# Autodesk Inventor assembly: Cam Follower
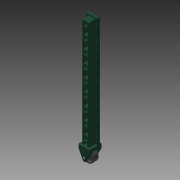
[picture p0: Inventor's stored thumbnail of the model, 180x180]
Saved by Autodesk Inventor 2016 SP2 (Build 200236200, 236)
## iProperties
Created: 2016-05-22
Part Number: Cam Follower
Document SubType Name: Assembly
Designer: Jacob
Author: Jacob
## Documents named in this file (4)
- D:\Users\Owner\Desktop\Inventor Files\VEX Parts\Imperial\Motion\Cam Follower.iam
- D:\Users\Owner\Desktop\Inventor Files\VEX Parts\Imperial\Motion\Components\Cam Follower Arm.ipt
- D:\Users\Owner\Desktop\Inventor Files\VEX Parts\Imperial\Motion\Components\Cam Follower Wheel.ipt
- D:\Users\Owner\Desktop\Inventor Files\VEX Parts\Imperial\Motion\Components\Cam Follower Pin.ipt
## Components (3 placed, 3 different names)
1. Cam Follower Arm:1 — Mate:1, Mate:2, Mate:3, Flush:1
2. Cam Follower Wheel:1 — Mate:1, Mate:2
3. Cam Follower Pin:1 — Mate:3, Flush:1
## Relationships (4: Mate 3, Flush 1)
- Mate:1 (0.1905 mm): Cam Follower Arm:1 ↔ Cam Follower Wheel:1
- Mate:2: Cam Follower Arm:1 ↔ Cam Follower Wheel:1
- Mate:3: Cam Follower Arm:1 ↔ Cam Follower Pin:1
- Flush:1: Cam Follower Arm:1 ↔ Cam Follower Pin:1
